# Autodesk Inventor assembly: assembly
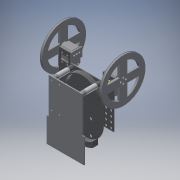
[picture p0: Inventor's stored thumbnail of the model, 180x180]
Saved by Autodesk Inventor 2016 (Build 200138000, 138)
## iProperties
Created: 2016-02-22
Part Number: assembly
Document SubType Name: Assembly
Designer: mkepler
Author: mkepler
## Documents named in this file (8)
- C:\Users\mkepler\Google Drive\Michael Kepler\College\ECE\ECE 590\Project 1\CAD files\assembly.iam
- C:\Users\mkepler\Google Drive\Michael Kepler\College\ECE\ECE 590\Project 1\CAD files\BaseChassis.ipt
- C:\Users\mkepler\Google Drive\Michael Kepler\College\ECE\ECE 590\Project 1\CAD files\Peg.ipt
- C:\Users\mkepler\Google Drive\Michael Kepler\College\ECE\ECE 590\Project 1\CAD files\TopChassis.ipt
- C:\Users\mkepler\Google Drive\Michael Kepler\College\ECE\ECE 492(3) Senior Design Project\ASL Robot Parts\Hand Final Design\xl-320 servo.ipt
- C:\Users\mkepler\Google Drive\Michael Kepler\College\ECE\ECE 590\Project 1\brace.ipt
- C:\Users\mkepler\Google Drive\Michael Kepler\College\ECE\ECE 590\Project 1\xl-320 servo.ipt
- C:\Users\mkepler\Google Drive\Michael Kepler\College\ECE\ECE 590\Project 1\CAD files\wheel.ipt
## Components (10 placed, 6 different names)
1. BaseChassis:1 — Insert:3, Mate:1, Mate:2, Insert:4, Mate:3, Insert:7, Insert:8
2. Peg:1 — Insert:3, Insert:6
3. Peg:2 — Mate:2, Mate:3, Insert:5
4. Peg:3 — Mate:1, Insert:4
5. TopChassis:1 — Insert:5, Insert:6
6. xl-320 servo:1 — Insert:9, Mate:4, Insert:12, Insert:14
7. brace:1 — Insert:7, Insert:8, Insert:9, Mate:4, Insert:10, Insert:11
8. xl-320 servo:2 — Insert:10, Insert:11, Insert:13, Insert:15
9. wheel:1 — Insert:12, Insert:14
10. wheel:2 — Insert:13, Insert:15
## Relationships (17: Insert 13, Mate 4)
- Insert:3: BaseChassis:1 ↔ Peg:1
- Mate:1: BaseChassis:1 ↔ Peg:3
- Mate:2: BaseChassis:1 ↔ Peg:2
- Insert:4: BaseChassis:1 ↔ Peg:3
- Mate:3: BaseChassis:1 ↔ Peg:2
- Insert:5: Peg:2 ↔ TopChassis:1
- Insert:6: Peg:1 ↔ TopChassis:1
- Insert:7: BaseChassis:1 ↔ brace:1
- Insert:8: BaseChassis:1 ↔ brace:1
- Insert:9: xl-320 servo:1 ↔ brace:1
- Mate:4: xl-320 servo:1 ↔ brace:1
- Insert:10: brace:1 ↔ xl-320 servo:2
- Insert:11: brace:1 ↔ xl-320 servo:2
- Insert:12: xl-320 servo:1 ↔ wheel:1
- Insert:13: xl-320 servo:2 ↔ wheel:2
- Insert:14: xl-320 servo:1 ↔ wheel:1
- Insert:15: xl-320 servo:2 ↔ wheel:2
